# Autodesk Inventor assembly: HalfRobotAssy
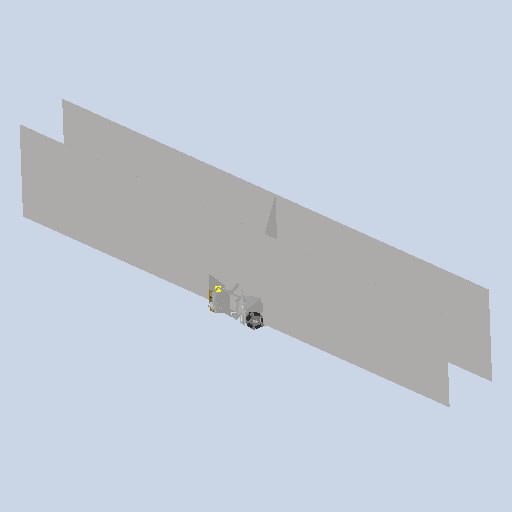
[picture p0: Inventor's stored thumbnail of the model, 512x512]
Saved by Autodesk Inventor 2025.1 (Build 291241000, 241)
## iProperties
Created: 2026-05-10
Part Number: HalfRobotAssy
Document SubType Name: Assembly
Designer: User
Author: User
## Documents named in this file (11)
- D:\One Drive\OneDrive - Politeknik Sultan Salahuddin Abdul Aziz Shah\Documents\Inventor\RobosotPSA\HalfRobotAssy.iam
- D:\One Drive\OneDrive - Politeknik Sultan Salahuddin Abdul Aziz Shah\Documents\Inventor\RobosotPSA\WheelMotor.iam
- D:\One Drive\OneDrive - Politeknik Sultan Salahuddin Abdul Aziz Shah\Documents\Inventor\RobosotPSA\FrontLeftCover.ipt
- D:\One Drive\OneDrive - Politeknik Sultan Salahuddin Abdul Aziz Shah\Documents\Inventor\RobosotPSA\MainBaseKicker_v2.ipt
- D:\One Drive\OneDrive - Politeknik Sultan Salahuddin Abdul Aziz Shah\Documents\Inventor\RobosotPSA\FrontRightCover.ipt
- D:\One Drive\OneDrive - Politeknik Sultan Salahuddin Abdul Aziz Shah\Documents\Inventor\RobosotPSA\BackCover.ipt
- D:\One Drive\OneDrive - Politeknik Sultan Salahuddin Abdul Aziz Shah\Documents\Inventor\RobosotPSA\CameraMount_v2.ipt
- D:\One Drive\OneDrive - Politeknik Sultan Salahuddin Abdul Aziz Shah\Documents\Inventor\RobosotPSA\TPLink_holder.ipt
- D:\One Drive\OneDrive - Politeknik Sultan Salahuddin Abdul Aziz Shah\Documents\Inventor\RobosotPSA\Assembly1.iam
- D:\One Drive\OneDrive - Politeknik Sultan Salahuddin Abdul Aziz Shah\Documents\Inventor\RobosotPSA\GripperAssy.iam
- D:\One Drive\OneDrive - Politeknik Sultan Salahuddin Abdul Aziz Shah\Documents\Inventor\RobosotPSA\Kicker_v2.ipt
## Components (13 placed, 10 different names)
1. WheelMotor:1 [sub-assembly] — Mate:1, Mate:2, Mate:3
2. WheelMotor:2 [sub-assembly] — Mate:7, Mate:8, Mate:9
3. WheelMotor:3 [sub-assembly] — Mate:4, Mate:5, Mate:6
4. WheelMotor:4 [sub-assembly] — Mate:10, Mate:11, Mate:12
5. FrontLeftCover:1 — Flush:1, Mate:13, Flush:2, Mate:19, Mate:20
6. MainBaseKicker_v2:1 — Mate:1, Mate:2, Mate:3, Mate:4, Mate:5, Mate:6, Mate:7, Mate:8, Mate:9, Mate:10, Mate:11, Mate:12, Flush:1, Mate:13, Flush:2, Mate:14, Flush:3, Mate:15, Mate:16, Mate:17, Mate:27, Mate:28, Mate:30
7. FrontRightCover:1 — Mate:14, Flush:3
8. BackCover:1 — Mate:15, Mate:16, Mate:17, Mate:18
9. CameraMount_v2:1 — Mate:18, Mate:19, Mate:20, Mate:21, Mate:22, Mate:23
10. TPLink_holder:1 — Mate:21, Mate:22, Mate:23, Mate:24, Mate:25, Mate:26
11. Assembly1:1 [sub-assembly] — Mate:24, Mate:25, Mate:26
12. GripperAssy:1 [sub-assembly] — Mate:31, Mate:32, Mate:33
13. Kicker_v2:1 — Mate:27, Mate:28, Mate:30, Mate:31, Mate:32, Mate:33
## Relationships (35: Mate 32, Flush 3)
- Mate:1: WheelMotor:1 ↔ MainBaseKicker_v2:1
- Mate:2: WheelMotor:1 ↔ MainBaseKicker_v2:1
- Mate:3: WheelMotor:1 ↔ MainBaseKicker_v2:1
- Mate:4: WheelMotor:3 ↔ MainBaseKicker_v2:1
- Mate:5: WheelMotor:3 ↔ MainBaseKicker_v2:1
- Mate:6: WheelMotor:3 ↔ MainBaseKicker_v2:1
- Mate:7: WheelMotor:2 ↔ MainBaseKicker_v2:1
- Mate:8: WheelMotor:2 ↔ MainBaseKicker_v2:1
- Mate:9: WheelMotor:2 ↔ MainBaseKicker_v2:1
- Mate:10: WheelMotor:4 ↔ MainBaseKicker_v2:1
- Mate:11: WheelMotor:4 ↔ MainBaseKicker_v2:1
- Mate:12: WheelMotor:4 ↔ MainBaseKicker_v2:1
- Flush:1: FrontLeftCover:1 ↔ MainBaseKicker_v2:1
- Mate:13 (0.231 mm): FrontLeftCover:1 ↔ MainBaseKicker_v2:1
- Flush:2: FrontLeftCover:1 ↔ MainBaseKicker_v2:1
- Mate:14 (0.231 mm): MainBaseKicker_v2:1 ↔ FrontRightCover:1
- Flush:3: MainBaseKicker_v2:1 ↔ FrontRightCover:1
- Mate:15 (0.231 mm): MainBaseKicker_v2:1 ↔ BackCover:1
- Mate:16: MainBaseKicker_v2:1 ↔ BackCover:1
- Mate:17: MainBaseKicker_v2:1 ↔ BackCover:1
- Mate:18: BackCover:1 ↔ CameraMount_v2:1
- Mate:19 (2 mm): FrontLeftCover:1 ↔ CameraMount_v2:1
- Mate:20 (3 mm): FrontLeftCover:1 ↔ CameraMount_v2:1
- Mate:21: CameraMount_v2:1 ↔ TPLink_holder:1
- Mate:22: CameraMount_v2:1 ↔ TPLink_holder:1
- Mate:23: CameraMount_v2:1 ↔ TPLink_holder:1
- Mate:24: TPLink_holder:1 ↔ Assembly1:1
- Mate:25: TPLink_holder:1 ↔ Assembly1:1
- Mate:26: TPLink_holder:1 ↔ Assembly1:1
- Mate:27: MainBaseKicker_v2:1 ↔ Kicker_v2:1
- Mate:28 (0.35 mm): MainBaseKicker_v2:1 ↔ Kicker_v2:1
- Mate:30 (11.685 mm): MainBaseKicker_v2:1 ↔ Kicker_v2:1
- Mate:31: GripperAssy:1 ↔ Kicker_v2:1
- Mate:32: GripperAssy:1 ↔ Kicker_v2:1
- Mate:33: GripperAssy:1 ↔ Kicker_v2:1
